# Autodesk Inventor assembly: RearZMotorMount
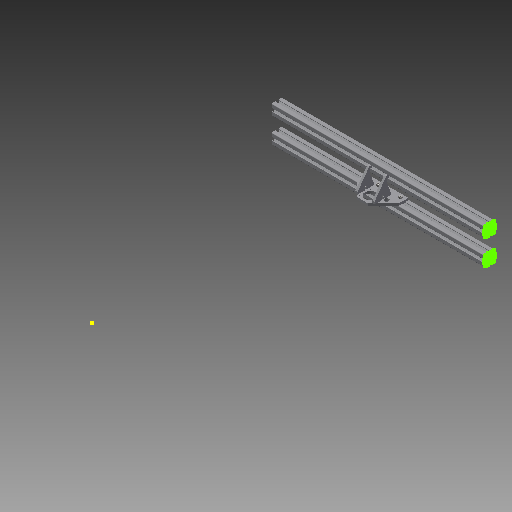
[picture p0: Inventor's stored thumbnail of the model, 512x512]
Saved by Autodesk Inventor 2017 (Build 210142000, 142)
## iProperties
Created: 2016-08-03
Part Number: RearZMotorMount
Document SubType Name: Assembly
Designer: User
Author: User
## Documents named in this file (4)
- C:\All INVENTOR\SL-Inventor\SL-Beast 3D Printer\RearZMotorMount.iam
- C:\All INVENTOR\SL-Inventor\SL-Beast 3D Printer\3030 600mm_CPY.ipt
- C:\All INVENTOR\SL-Inventor\SL-Beast 3D Printer\Z Motor Mount.iam
- C:\All INVENTOR\SL-Inventor\SL-Beast 3D Printer\Lower Panels.iam
## Components (4 placed, 3 different names)
1. 3030 600mm_CPY:1
2. 3030 600mm_CPY:2
3. Z Motor Mount:1 [sub-assembly]
4. Lower Panels:1 [sub-assembly]
## Relationships (3: Flush 1, Angle 1, Mate 1)
- [Flush]: 3030 600mm_CPY:1 ↔ Lower Panels:1
- [Angle] (180 deg): 3030 600mm_CPY:2 ↔ Z Motor Mount:1
- [Mate]: 3030 600mm_CPY:1 ↔ Lower Panels:1
